# Autodesk Inventor assembly: 42146-20-01
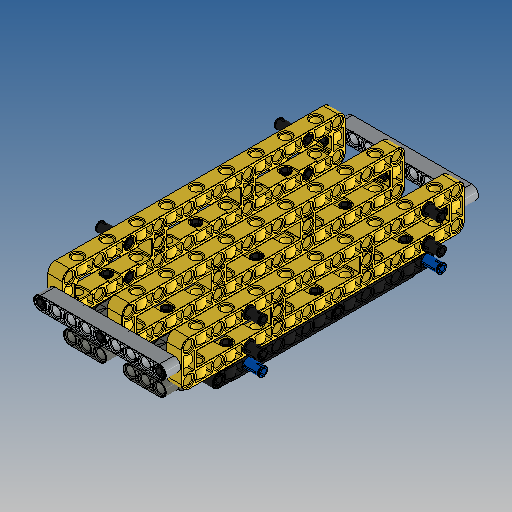
[picture p0: Inventor's stored thumbnail of the model, 512x512]
Saved by Autodesk Inventor 2025 (Build 290162010, 162A)
## iProperties
Created: 2024-11-22
Part Number: 42146-20-01
Material: Generisch
Document SubType Name: Assembly
Designer: hp.muther
Author: hp.muther
## Documents named in this file (9)
- D:\Inventor\Projekte\Muther\LEGO Technic\LEGO Technik - Raupenkran LR 13000 (42146)\42146-01-20-01.iam
- D:\Inventor\Projekte\Muther\LEGO Technic\LEGO Pieces\Lochbalken\771710-Black.ipt
- D:\Inventor\Projekte\Muther\LEGO Technic\LEGO Pieces\Pin's\6558-Blue.ipt
- D:\Inventor\Projekte\Muther\LEGO Technic\LEGO Pieces\Lochbalken\32523-Yellow.ipt
- D:\Inventor\Projekte\Muther\LEGO Technic\LEGO Pieces\Paneelen\15458-Yellow.ipt
- D:\Inventor\Projekte\Muther\LEGO Technic\LEGO Pieces\Paneelen\71709-DkBluishGray.ipt
- D:\Inventor\Projekte\Muther\LEGO Technic\LEGO Pieces\Pin's\2780-Black.ipt
- D:\Inventor\Projekte\Muther\LEGO Technic\LEGO Pieces\Rahmen, T-Stücke\67491-Yellow.ipt
- D:\Inventor\Projekte\Muther\LEGO Technic\LEGO Pieces\Lochbalken\40490-LtBluishGray.ipt
## Components (53 placed, 8 different names)
1. 771710-Black:1 — Einfügen:1, Einfügen:2, Einfügen:3, Einfügen:4, Einfügen:9, Einfügen:14, Einfügen:28, Einfügen:29, Einfügen:30, Einfügen:48
2. 6558-Blue:1 — Einfügen:2
3. 6558-Blue:2 — Einfügen:1, Passend:3, Passend:6
4. 6558-Blue:3 — Einfügen:3
5. 6558-Blue:4 — Einfügen:4
6. 6558-Blue:5 — Einfügen:6, Passend:1
7. 6558-Blue:6 — Einfügen:5, Passend:2
8. 32523-Yellow:1 — Einfügen:5, Einfügen:6, Einfügen:7, Einfügen:8
9. 15458-Yellow:1 — Einfügen:7, Einfügen:9, Passend:1, Einfügen:23
10. 71709-DkBluishGray:1 — Einfügen:8, Passend:2, Passend:3, Passend:8
11. 6558-Blue:7
12. 6558-Blue:8
13. 32523-Yellow:2
14. 15458-Yellow:2 — Einfügen:14, Einfügen:24
15. 71709-DkBluishGray:2 — Passend:6, Passend:7
16. 2780-Black:1 — Einfügen:18, Passend:8
17. 2780-Black:2 — Einfügen:17
18. 771710-Black:2 — Einfügen:17, Einfügen:18, Einfügen:23, Einfügen:31, Einfügen:32, Einfügen:33, Einfügen:49
19. 6558-Blue:11
20. 6558-Blue:12
21. 2780-Black:3 — Einfügen:31, Passend:11
22. 2780-Black:4 — Einfügen:30, Passend:10
23. 2780-Black:5 — Einfügen:28
24. 2780-Black:6 — Einfügen:33
25. 2780-Black:7 — Einfügen:32
26. 2780-Black:8 — Einfügen:29
27. 2780-Black:9 — Einfügen:27, Passend:9
28. 2780-Black:10 — Einfügen:26
29. 2780-Black:11 — Einfügen:25
30. 2780-Black:12 — Passend:7
31. 2780-Black:13
32. 771710-Black:3 — Einfügen:24, Einfügen:26, Einfügen:27, Einfügen:25, Einfügen:50
33. 6558-Blue:13
34. 6558-Blue:14
35. 2780-Black:14 — Einfügen:39
36. 2780-Black:15 — Einfügen:38
37. 2780-Black:16 — Einfügen:37
38. 2780-Black:17 — Einfügen:35, Passend:12
39. 2780-Black:18 — Einfügen:36
40. 2780-Black:19 — Einfügen:34, Passend:13
41. 67491-Yellow:1 — Einfügen:34, Einfügen:35, Einfügen:36, Einfügen:37, Einfügen:38, Einfügen:39, Einfügen:49, Passend:11
42. 2780-Black:20 — Einfügen:45
43. 2780-Black:21 — Einfügen:44
44. 2780-Black:22
45. 2780-Black:23
46. 2780-Black:24
47. 2780-Black:25
48. 67491-Yellow:2 — Einfügen:44, Einfügen:45, Einfügen:50, Passend:9, Einfügen:51, Einfügen:52
49. 2780-Black:26
50. 2780-Black:27
51. 67491-Yellow:3 — Einfügen:48, Passend:10
52. 40490-LtBluishGray:1 — Einfügen:52, Passend:12
53. 40490-LtBluishGray:2 — Einfügen:51, Passend:13
## Relationships (65: Insert 52, Mate 13)
- Einfügen:1 [Insert]: 771710-Black:1 ↔ 6558-Blue:2
- Einfügen:2 [Insert]: 771710-Black:1 ↔ 6558-Blue:1
- Einfügen:3 [Insert]: 771710-Black:1 ↔ 6558-Blue:3
- Einfügen:4 [Insert]: 771710-Black:1 ↔ 6558-Blue:4
- Einfügen:5 [Insert]: 6558-Blue:6 ↔ 32523-Yellow:1
- Einfügen:6 [Insert]: 6558-Blue:5 ↔ 32523-Yellow:1
- Einfügen:7 [Insert]: 32523-Yellow:1 ↔ 15458-Yellow:1
- Einfügen:8 [Insert]: 32523-Yellow:1 ↔ 71709-DkBluishGray:1
- Einfügen:9 [Insert]: 771710-Black:1 ↔ 15458-Yellow:1
- Passend:1 [Mate]: 6558-Blue:5 ↔ 15458-Yellow:1
- Passend:2 [Mate]: 6558-Blue:6 ↔ 71709-DkBluishGray:1
- Passend:3 [Mate]: 6558-Blue:2 ↔ 71709-DkBluishGray:1
- [Insert]: 6558-Blue:8 ↔ 32523-Yellow:2
- [Insert]: 6558-Blue:7 ↔ 32523-Yellow:2
- [Insert]: 32523-Yellow:2 ↔ 15458-Yellow:2
- [Insert]: 32523-Yellow:2 ↔ 71709-DkBluishGray:2
- [Mate]: 6558-Blue:7 ↔ 15458-Yellow:2
- [Mate]: 6558-Blue:8 ↔ 71709-DkBluishGray:2
- Einfügen:14 [Insert]: 771710-Black:1 ↔ 15458-Yellow:2
- Passend:6 [Mate]: 6558-Blue:2 ↔ 71709-DkBluishGray:2
- [Insert]: 771710-Black:2 ↔ 6558-Blue:11
- [Insert]: 771710-Black:2 ↔ 6558-Blue:12
- Einfügen:17 [Insert]: 2780-Black:2 ↔ 771710-Black:2
- Einfügen:18 [Insert]: 2780-Black:1 ↔ 771710-Black:2
- [Insert]: 771710-Black:3 ↔ 6558-Blue:13
- [Insert]: 771710-Black:3 ↔ 6558-Blue:14
- [Insert]: 2780-Black:13 ↔ 771710-Black:3
- [Insert]: 2780-Black:12 ↔ 771710-Black:3
- Einfügen:23 [Insert]: 15458-Yellow:1 ↔ 771710-Black:2
- Einfügen:24 [Insert]: 15458-Yellow:2 ↔ 771710-Black:3
- Passend:7 [Mate]: 71709-DkBluishGray:2 ↔ 2780-Black:12
- Passend:8 [Mate]: 71709-DkBluishGray:1 ↔ 2780-Black:1
- Einfügen:25 [Insert]: 2780-Black:11 ↔ 771710-Black:3
- Einfügen:26 [Insert]: 2780-Black:10 ↔ 771710-Black:3
- Einfügen:27 [Insert]: 2780-Black:9 ↔ 771710-Black:3
- Einfügen:28 [Insert]: 771710-Black:1 ↔ 2780-Black:5
- Einfügen:29 [Insert]: 771710-Black:1 ↔ 2780-Black:8
- Einfügen:30 [Insert]: 771710-Black:1 ↔ 2780-Black:4
- Einfügen:31 [Insert]: 771710-Black:2 ↔ 2780-Black:3
- Einfügen:32 [Insert]: 771710-Black:2 ↔ 2780-Black:7
- Einfügen:33 [Insert]: 771710-Black:2 ↔ 2780-Black:6
- Einfügen:34 [Insert]: 2780-Black:19 ↔ 67491-Yellow:1
- Einfügen:35 [Insert]: 2780-Black:17 ↔ 67491-Yellow:1
- Einfügen:36 [Insert]: 2780-Black:18 ↔ 67491-Yellow:1
- Einfügen:37 [Insert]: 2780-Black:16 ↔ 67491-Yellow:1
- Einfügen:38 [Insert]: 2780-Black:15 ↔ 67491-Yellow:1
- Einfügen:39 [Insert]: 2780-Black:14 ↔ 67491-Yellow:1
- [Insert]: 2780-Black:25 ↔ 67491-Yellow:2
- [Insert]: 2780-Black:23 ↔ 67491-Yellow:2
- [Insert]: 2780-Black:24 ↔ 67491-Yellow:2
- [Insert]: 2780-Black:22 ↔ 67491-Yellow:2
- Einfügen:44 [Insert]: 2780-Black:21 ↔ 67491-Yellow:2
- Einfügen:45 [Insert]: 2780-Black:20 ↔ 67491-Yellow:2
- [Insert]: 2780-Black:27 ↔ 67491-Yellow:3
- [Insert]: 2780-Black:26 ↔ 67491-Yellow:3
- Einfügen:48 [Insert]: 771710-Black:1 ↔ 67491-Yellow:3
- Einfügen:49 [Insert]: 771710-Black:2 ↔ 67491-Yellow:1
- Einfügen:50 [Insert]: 771710-Black:3 ↔ 67491-Yellow:2
- Passend:9 [Mate]: 2780-Black:9 ↔ 67491-Yellow:2
- Passend:10 [Mate]: 2780-Black:4 ↔ 67491-Yellow:3
- Passend:11 [Mate]: 2780-Black:3 ↔ 67491-Yellow:1
- Einfügen:51 [Insert]: 67491-Yellow:2 ↔ 40490-LtBluishGray:2
- Einfügen:52 [Insert]: 67491-Yellow:2 ↔ 40490-LtBluishGray:1
- Passend:12 [Mate]: 2780-Black:17 ↔ 40490-LtBluishGray:1
- Passend:13 [Mate]: 2780-Black:19 ↔ 40490-LtBluishGray:2
## Named parameters: d12_d7 = 0 mm, d13_d9 = 0 mm, d14_d10 = 0 mm, d15_d4 = 0 mm, d16_d5 = 0 mm, d17_d6 = 0 mm, d20_d3 = 0 mm, d21_d1 = 0 mm, d24_d20_d3 = 0 mm, d25_d21_d1 = 0 mm, d26_d22 = 0 mm, d27_d23 = 0 mm, d47_d42 = 0 mm, d48_d43 = 0 mm, d49_d44 = 0 mm, d50_d45 = 0 mm, d51_d46 = 0 mm, d52_d41 = 0 mm, d53_d47_d42 = 0 mm, d54_d52_d41 = 0 mm
